# Autodesk Inventor assembly: Assembly_Cube_Syringepump_Micro_v3
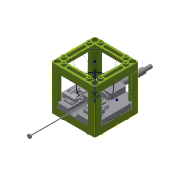
[picture p0: Inventor's stored thumbnail of the model, 180x180]
Saved by Autodesk Inventor 2022 (Build 260153000, 153)
## iProperties
Created: 2020-11-11
Part Number: Assembly_Cube_Syringepump_Micro_v3
Document SubType Name: Assembly
Designer: marsikovabarbora
Author: marsikovabarbora
## Documents named in this file (7)
- C:\Users\diederichbenedict\Dropbox\Dokumente\Promotion\PROJECTS\UC2\02_CAD\INVENTOR\uc2_v3\Assembly_Cube_Syringepump_Micro_v3.iam
- C:\Users\diederichbenedict\Dropbox\Dokumente\Promotion\PROJECTS\UC2\02_CAD\INVENTOR\uc2_v3\Assembly_Cube_empty_IM_v3.iam
- C:\Users\diederichbenedict\Dropbox\Dokumente\Promotion\PROJECTS\UC2\02_CAD\INVENTOR\uc2_v3\00_Syringe_10ml.ipt
- C:\Users\diederichbenedict\Dropbox\Dokumente\Promotion\PROJECTS\UC2\02_CAD\INVENTOR\uc2_v3\00_Microlinearmotor_aliexpress_5mm.ipt
- C:\Users\diederichbenedict\Dropbox\Dokumente\Promotion\PROJECTS\UC2\02_CAD\INVENTOR\uc2_v3\20_Cube_Insert_Template_magnetic_clamp_v3.ipt
- C:\Users\diederichbenedict\Dropbox\Dokumente\Promotion\PROJECTS\UC2\02_CAD\INVENTOR\uc2_v3\20_Cube_Insert_Syringepump_Micro_v3.ipt
- C:\Users\diederichbenedict\Dropbox\Dokumente\Promotion\PROJECTS\UC2\02_CAD\INVENTOR\uc2_v3\20_Cube_Insert_Syringepump_Micro_syringeclamp_v3.ipt
## Components (7 placed, 6 different names)
1. Assembly_Cube_empty_IM_v3:1 [sub-assembly] — Mate:1, Mate:2, Mate:3, Passend:8, Passend:9, Passend:10, Passend:11, Fluchtend:1
2. 20_Cube_Insert_Syringepump_Micro_v3:1 — Passend:8, Passend:9, Passend:10, Fluchtend:13, Passend:12, Fluchtend:14, Fluchtend:15, Fluchtend:16, Fluchtend:17, Passend:19, Passend:20
3. 00_Syringe_10ml:1 — Passend:11, Fluchtend:1, Fluchtend:13, Fluchtend:20
4. 00_Microlinearmotor_aliexpress_5mm:1 — Passend:12, Fluchtend:14, Fluchtend:15, Fluchtend:18
5. 20_Cube_Insert_Template_magnetic_clamp_v3:1 — Fluchtend:16, Fluchtend:17
6. 00_Microlinearmotor_aliexpress_5mm:2 — Passend:19, Fluchtend:18, Passend:20, Fluchtend:19
7. 20_Cube_Insert_Syringepump_Micro_syringeclamp_v3:1 — Fluchtend:19, Fluchtend:20
## Relationships (19: Mate 10, Flush 9)
- Mate:1: Assembly_Cube_empty_IM_v3:1
- Mate:2: Assembly_Cube_empty_IM_v3:1
- Mate:3: Assembly_Cube_empty_IM_v3:1
- Passend:8 [Mate]: Assembly_Cube_empty_IM_v3:1 ↔ 20_Cube_Insert_Syringepump_Micro_v3:1
- Passend:9 [Mate]: Assembly_Cube_empty_IM_v3:1 ↔ 20_Cube_Insert_Syringepump_Micro_v3:1
- Passend:10 [Mate]: Assembly_Cube_empty_IM_v3:1 ↔ 20_Cube_Insert_Syringepump_Micro_v3:1
- Passend:11 [Mate]: Assembly_Cube_empty_IM_v3:1 ↔ 00_Syringe_10ml:1
- Fluchtend:1 [Flush] (-30 mm): Assembly_Cube_empty_IM_v3:1 ↔ 00_Syringe_10ml:1
- Fluchtend:13 [Flush]: 20_Cube_Insert_Syringepump_Micro_v3:1 ↔ 00_Syringe_10ml:1
- Passend:12 [Mate]: 20_Cube_Insert_Syringepump_Micro_v3:1 ↔ 00_Microlinearmotor_aliexpress_5mm:1
- Fluchtend:14 [Flush] (5 mm): 20_Cube_Insert_Syringepump_Micro_v3:1 ↔ 00_Microlinearmotor_aliexpress_5mm:1
- Fluchtend:15 [Flush] (8 mm): 20_Cube_Insert_Syringepump_Micro_v3:1 ↔ 00_Microlinearmotor_aliexpress_5mm:1
- Fluchtend:16 [Flush]: 20_Cube_Insert_Syringepump_Micro_v3:1 ↔ 20_Cube_Insert_Template_magnetic_clamp_v3:1
- Fluchtend:17 [Flush]: 20_Cube_Insert_Syringepump_Micro_v3:1 ↔ 20_Cube_Insert_Template_magnetic_clamp_v3:1
- Passend:19 [Mate]: 20_Cube_Insert_Syringepump_Micro_v3:1 ↔ 00_Microlinearmotor_aliexpress_5mm:2
- Fluchtend:18 [Flush]: 00_Microlinearmotor_aliexpress_5mm:1 ↔ 00_Microlinearmotor_aliexpress_5mm:2
- Passend:20 [Mate] (1.4 mm): 20_Cube_Insert_Syringepump_Micro_v3:1 ↔ 00_Microlinearmotor_aliexpress_5mm:2
- Fluchtend:19 [Flush]: 00_Microlinearmotor_aliexpress_5mm:2 ↔ 20_Cube_Insert_Syringepump_Micro_syringeclamp_v3:1
- Fluchtend:20 [Flush]: 00_Syringe_10ml:1 ↔ 20_Cube_Insert_Syringepump_Micro_syringeclamp_v3:1
